# Autodesk Inventor assembly: Passive Intake Arm
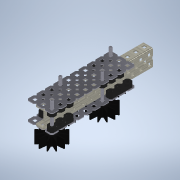
[picture p0: Inventor's stored thumbnail of the model, 180x180]
Saved by Autodesk Inventor 2020 (Build 240168000, 168)
## iProperties
Created: 2019-09-18
Part Number: Passive Intake Arm
Document SubType Name: Assembly
Designer: Corey
Author: Corey
## Documents named in this file (6)
- C:\Users\Corey\Documents\Tower-Takeover-CAD\Parts\Center Arm Intake.iam
- C:\Users\Corey\Documents\Tower-Takeover-CAD\Parts\Structure\C-Channels\Aluminum\2-Wide\Aluminum C-Channel 1x2x1x35.ipt
- C:\Users\Corey\Documents\Tower-Takeover-CAD\Parts\Motion\Wheels & Rollers\Intake Roller.ipt
- C:\Users\Corey\Documents\Tower-Takeover-CAD\Parts\Motion\Bearing Flat.ipt
- C:\Users\Corey\Documents\Tower-Takeover-CAD\Parts\Motion\Drive Shafts\Drive Shaft 2''.ipt
- C:\Users\Corey\Documents\Tower-Takeover-CAD\Parts\Structure\Plates\Plate 5x3.ipt
## Components (21 placed, 5 different names)
1. Aluminum C-Channel 1x2x1x35:1 — Mate:11, Flush:1, Flush:2, Mate:12, Flush:3, Flush:4, Mate:13, Mate:14, Flush:5, Flush:6, Flush:7, Flush:8
2. Intake Roller:1
3. Intake Roller:2
4. Bearing Flat:1 — Mate:15, Insert:29, Insert:30
5. Bearing Flat:2 — Mate:18, Insert:17, Insert:18
6. Bearing Flat:3 — Mate:16, Insert:13, Insert:14
7. Bearing Flat:4 — Mate:17, Insert:31, Insert:32
8. Drive Shaft 2'':1
9. Drive Shaft 2'':2
10. Plate 5x3:1 — Mate:13, Flush:5, Flush:6, Mate:17, Mate:19, Insert:19, Insert:20, Insert:31, Insert:32, Mate:25
11. Plate 5x3:2 — Mate:14, Flush:7, Flush:8, Mate:18, Insert:17, Insert:18, Mate:20, Mate:28
12. Plate 5x3:3 — Mate:12, Flush:3, Flush:4, Mate:16, Insert:13, Insert:14, Mate:22, Insert:33, Insert:34
13. Plate 5x3:4 — Mate:11, Flush:1, Flush:2, Mate:15, Mate:21, Insert:21, Insert:22, Insert:29, Insert:30
14. Bearing Flat:5 — Mate:20
15. Bearing Flat:6 — Mate:19, Insert:19, Insert:20
16. Bearing Flat:7 — Mate:21, Insert:21, Insert:22, Insert:27
17. Bearing Flat:8 — Mate:22, Insert:28, Insert:33, Insert:34
18. Drive Shaft 2'':3 — Insert:27, Mate:23, Mate:24
19. Drive Shaft 2'':4 — Insert:28, Mate:26, Mate:27
20. Intake Roller:3 — Mate:23, Mate:24, Mate:25
21. Intake Roller:4 — Mate:26, Mate:27, Mate:28
## Relationships (50: Mate 24, Insert 18, Flush 8)
- [Insert] (-12.7 mm): Bearing Flat:1 ↔ Drive Shaft 2'':1
- [Insert] (-12.7 mm): Bearing Flat:3 ↔ Drive Shaft 2'':2
- [Mate]: Intake Roller:1 ↔ Drive Shaft 2'':1
- [Mate]: Intake Roller:1 ↔ Drive Shaft 2'':1
- [Mate] (2.54 mm): Aluminum C-Channel 1x2x1x35:1 ↔ Intake Roller:1
- [Mate]: Intake Roller:2 ↔ Drive Shaft 2'':2
- [Mate]: Intake Roller:2 ↔ Drive Shaft 2'':2
- [Mate] (2.54 mm): Aluminum C-Channel 1x2x1x35:1 ↔ Intake Roller:2
- Mate:11: Aluminum C-Channel 1x2x1x35:1 ↔ Plate 5x3:4
- Flush:1: Aluminum C-Channel 1x2x1x35:1 ↔ Plate 5x3:4
- Flush:2: Aluminum C-Channel 1x2x1x35:1 ↔ Plate 5x3:4
- Mate:12: Aluminum C-Channel 1x2x1x35:1 ↔ Plate 5x3:3
- Flush:3: Aluminum C-Channel 1x2x1x35:1 ↔ Plate 5x3:3
- Flush:4: Aluminum C-Channel 1x2x1x35:1 ↔ Plate 5x3:3
- Mate:13: Aluminum C-Channel 1x2x1x35:1 ↔ Plate 5x3:1
- Mate:14: Aluminum C-Channel 1x2x1x35:1 ↔ Plate 5x3:2
- Flush:5: Aluminum C-Channel 1x2x1x35:1 ↔ Plate 5x3:1
- Flush:6: Aluminum C-Channel 1x2x1x35:1 ↔ Plate 5x3:1
- Flush:7: Aluminum C-Channel 1x2x1x35:1 ↔ Plate 5x3:2
- Flush:8: Aluminum C-Channel 1x2x1x35:1 ↔ Plate 5x3:2
- Mate:15: Bearing Flat:1 ↔ Plate 5x3:4
- Mate:16: Bearing Flat:3 ↔ Plate 5x3:3
- Insert:13: Bearing Flat:3 ↔ Plate 5x3:3
- Insert:14: Bearing Flat:3 ↔ Plate 5x3:3
- Mate:17: Bearing Flat:4 ↔ Plate 5x3:1
- Mate:18: Bearing Flat:2 ↔ Plate 5x3:2
- Insert:17: Bearing Flat:2 ↔ Plate 5x3:2
- Insert:18: Bearing Flat:2 ↔ Plate 5x3:2
- Mate:19: Plate 5x3:1 ↔ Bearing Flat:6
- Mate:20: Plate 5x3:2 ↔ Bearing Flat:5
- Mate:21: Plate 5x3:4 ↔ Bearing Flat:7
- Mate:22: Plate 5x3:3 ↔ Bearing Flat:8
- Insert:19: Plate 5x3:1 ↔ Bearing Flat:6
- Insert:20: Plate 5x3:1 ↔ Bearing Flat:6
- Insert:21: Plate 5x3:4 ↔ Bearing Flat:7
- Insert:22: Plate 5x3:4 ↔ Bearing Flat:7
- Insert:27 (-12.7 mm): Bearing Flat:7 ↔ Drive Shaft 2'':3
- Insert:28 (-12.7 mm): Bearing Flat:8 ↔ Drive Shaft 2'':4
- Insert:29: Bearing Flat:1 ↔ Plate 5x3:4
- Insert:30: Bearing Flat:1 ↔ Plate 5x3:4
- Insert:31: Bearing Flat:4 ↔ Plate 5x3:1
- Insert:32: Bearing Flat:4 ↔ Plate 5x3:1
- Mate:23: Drive Shaft 2'':3 ↔ Intake Roller:3
- Mate:24: Drive Shaft 2'':3 ↔ Intake Roller:3
- Mate:25 (1.27 mm): Plate 5x3:1 ↔ Intake Roller:3
- Insert:33: Plate 5x3:3 ↔ Bearing Flat:8
- Insert:34: Plate 5x3:3 ↔ Bearing Flat:8
- Mate:26: Drive Shaft 2'':4 ↔ Intake Roller:4
- Mate:27: Drive Shaft 2'':4 ↔ Intake Roller:4
- Mate:28 (1.27 mm): Plate 5x3:2 ↔ Intake Roller:4
